# Autodesk Inventor assembly: Mecanum_Assembly
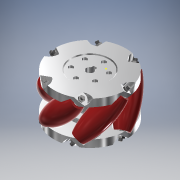
[picture p0: Inventor's stored thumbnail of the model, 180x180]
Saved by Autodesk Inventor 2018 (Build 220112000, 112)
## iProperties
Created: 2017-09-05
Part Number: Mecanum_Assembly
Document SubType Name: Assembly
Designer: P136265
Author: P136265
## Documents named in this file (9)
- C:\Users\p447144\Documents\mecanum-cad\Mecanum_Assembly.iam
- C:\Users\p447144\Documents\mecanum-cad\roller 8-19-6 bearing.ipt
- C:\Users\p447144\Documents\Inventor\Content Center Files\R2018\en-US\DIN 625 SKF(4)\DIN 625 SKF - SKF 619_8-2Z.ipt
- C:\Users\p447144\Documents\mecanum-cad\MecanumShaft.ipt
- C:\Users\p447144\Documents\mecanum-cad\PE_Sleeve.ipt
- C:\Users\p447144\Documents\mecanum-cad\CheekPlate.ipt
- C:\Users\p447144\Documents\mecanum-cad\MecanumHub.ipt
- C:\Users\p447144\Documents\mecanum-cad\Washer.ipt
- C:\Users\p447144\Documents\Inventor\Content Center Files\R2018\en-US\BS 4183(1)\BS 4183 - M8(1).ipt
## Components (57 placed, 8 different names)
1. CheekPlate:1 — Angle:10, Angle:11, Mate:19, Angle:12, Mate:20, Mate:21, Angle:13, Angle:14, Mate:25
2. MecanumHub:1 — Angle:12, Mate:20, Mate:21, Mate:22
3. CheekPlate:2 — Angle:13, Angle:14, Angle:15, Mate:22, Mate:23, Mate:27
4. roller 8-19-6 bearing:1 — Mate:1, Angle:1, Mate:2, Angle:11
5. BS 4183 - Metric M8:1 — Mate:24, Mate:25
6. BS 4183 - Metric M8:7 — Mate:26, Mate:27
7. roller 8-19-6 bearing:2
8. BS 4183 - Metric M8:2
9. BS 4183 - Metric M8:8
10. roller 8-19-6 bearing:3 — Insert:1, Insert:2, Angle:8, Angle:9
11. BS 4183 - Metric M8:3
12. BS 4183 - Metric M8:9
13. roller 8-19-6 bearing:4 — Angle:2, Mate:3, Mate:4
14. BS 4183 - Metric M8:4
15. BS 4183 - Metric M8:10
16. roller 8-19-6 bearing:5
17. BS 4183 - Metric M8:5
18. BS 4183 - Metric M8:11
19. roller 8-19-6 bearing:6
20. BS 4183 - Metric M8:6
21. BS 4183 - Metric M8:12
22. DIN 625 SKF- with two Z shields SKF 619/8-2Z:1 — Insert:1, Mate:17
23. DIN 625 SKF- with two Z shields SKF 619/8-2Z:3
24. DIN 625 SKF- with two Z shields SKF 619/8-2Z:4
25. DIN 625 SKF- with two Z shields SKF 619/8-2Z:5
26. DIN 625 SKF- with two Z shields SKF 619/8-2Z:6
27. DIN 625 SKF- with two Z shields SKF 619/8-2Z:7
28. DIN 625 SKF- with two Z shields SKF 619/8-2Z:2 — Insert:2, Mate:15
29. DIN 625 SKF- with two Z shields SKF 619/8-2Z:8 — Flush:1
30. DIN 625 SKF- with two Z shields SKF 619/8-2Z:9
31. DIN 625 SKF- with two Z shields SKF 619/8-2Z:10
32. DIN 625 SKF- with two Z shields SKF 619/8-2Z:11
33. DIN 625 SKF- with two Z shields SKF 619/8-2Z:12
34. MecanumShaft:1 — Angle:2, Mate:3, Flush:1, Angle:3, Angle:15, Mate:23
35. MecanumShaft:2 — Mate:24, Mate:26
36. MecanumShaft:3
37. MecanumShaft:4
38. MecanumShaft:5
39. MecanumShaft:6 — Mate:16, Mate:18, Angle:10
40. PE_Sleeve:1 — Angle:3, Mate:4
41. PE_Sleeve:2
42. PE_Sleeve:3
43. PE_Sleeve:4
44. PE_Sleeve:5
45. PE_Sleeve:6
46. Washer:2 — Angle:9, Mate:17, Mate:18
47. Washer:1 — Angle:8, Mate:15, Mate:16
48. Washer:3
49. Washer:4
50. Washer:5
51. Washer:6
52. Washer:7
53. Washer:8
54. Washer:9 — Mate:19
55. Washer:10
56. Washer:11
57. Washer:12
## Component patterns: (6 elements, first: roller 8-19-6 bearing:1 + BS 4183 - Metric M8:1 + BS 4183 - Metric M8:7), (6 elements, first: DIN 625 SKF- with two Z shields SKF 619/8-2Z:1), (6 elements, first: DIN 625 SKF- with two Z shields SKF 619/8-2Z:2), (6 elements, first: MecanumShaft:1), (6 elements, first: PE_Sleeve:1), (6 elements, first: Washer:2 + Washer:1)
## Relationships (31: Mate 17, Angle 11, Insert 2, Flush 1)
- Mate:1 (75 mm): roller 8-19-6 bearing:1
- Angle:1 (45 deg): roller 8-19-6 bearing:1
- Mate:2: roller 8-19-6 bearing:1
- Insert:1: roller 8-19-6 bearing:3 ↔ DIN 625 SKF- with two Z shields SKF 619/8-2Z:1
- Insert:2: roller 8-19-6 bearing:3 ↔ DIN 625 SKF- with two Z shields SKF 619/8-2Z:2
- Angle:2 (0 deg): roller 8-19-6 bearing:4 ↔ MecanumShaft:1
- Mate:3: roller 8-19-6 bearing:4 ↔ MecanumShaft:1
- Flush:1 (-20 mm): DIN 625 SKF- with two Z shields SKF 619/8-2Z:8 ↔ MecanumShaft:1
- Angle:3 (0 deg): MecanumShaft:1 ↔ PE_Sleeve:1
- Mate:4: roller 8-19-6 bearing:4 ↔ PE_Sleeve:1
- Angle:8 (0 deg): roller 8-19-6 bearing:3 ↔ Washer:1
- Mate:15: DIN 625 SKF- with two Z shields SKF 619/8-2Z:2 ↔ Washer:1
- Mate:16: MecanumShaft:6 ↔ Washer:1
- Angle:9 (0 deg): roller 8-19-6 bearing:3 ↔ Washer:2
- Mate:17: DIN 625 SKF- with two Z shields SKF 619/8-2Z:1 ↔ Washer:2
- Mate:18: MecanumShaft:6 ↔ Washer:2
- Angle:10 (0 deg): CheekPlate:1 ↔ MecanumShaft:6
- Angle:11 (0 deg): CheekPlate:1 ↔ roller 8-19-6 bearing:1
- Mate:19: CheekPlate:1 ↔ Washer:9
- Angle:12 (0 deg): CheekPlate:1 ↔ MecanumHub:1
- Mate:20: CheekPlate:1 ↔ MecanumHub:1
- Mate:21: CheekPlate:1 ↔ MecanumHub:1
- Angle:13 (0 deg): CheekPlate:1 ↔ CheekPlate:2
- Angle:14 (0 deg): CheekPlate:1 ↔ CheekPlate:2
- Angle:15 (0 deg): CheekPlate:2 ↔ MecanumShaft:1
- Mate:22: MecanumHub:1 ↔ CheekPlate:2
- Mate:23: CheekPlate:2 ↔ MecanumShaft:1
- Mate:24: BS 4183 - Metric M8:1 ↔ MecanumShaft:2
- Mate:25: CheekPlate:1 ↔ BS 4183 - Metric M8:1
- Mate:26: BS 4183 - Metric M8:7 ↔ MecanumShaft:2
- Mate:27: CheekPlate:2 ↔ BS 4183 - Metric M8:7
